# Autodesk Inventor assembly: radio on stand
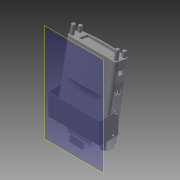
[picture p0: Inventor's stored thumbnail of the model, 180x180]
Saved by Autodesk Inventor 2014 (Build 180170000, 170)
## iProperties
Created: 2014-04-06
Part Number: radio on stand
Document SubType Name: Assembly
Designer: Tyler
Author: Tyler
## Documents named in this file (6)
- C:\Users\Tyler\Documents\ft8900cad\radio on stand.iam
- C:\Users\Tyler\Documents\ft8900cad\radio_base.ipt
- C:\Users\Tyler\Documents\ft8900cad\radio.ipt
- C:\Users\Tyler\Documents\Inventor\Content Center Files\R2014\en-US\GB_T 2671.1-2004\Screw GB_T 2171.1 M4 x 6.ipt
- C:\Users\Tyler\Documents\ft8900cad\controlunit.iam
- C:\Users\Tyler\Documents\ft8900cad\radio_head.ipt
## Components (8 placed, 5 different names)
1. radio_base:1 — Insert:1, Insert:2, Insert:3, Insert:4, Insert:5, Insert:6, Mate:2, Flush:3, Flush:4
2. radio:1 — Insert:1, Insert:2, Mate:1, Flush:1, Flush:2
3. Screw GB/T 2671.1-2004 M4x6 Property Class 4.8:1 — Insert:3
4. Screw GB/T 2671.1-2004 M4x6 Property Class 4.8:2 — Insert:4
5. Screw GB/T 2671.1-2004 M4x6 Property Class 4.8:3 — Insert:5
6. Screw GB/T 2671.1-2004 M4x6 Property Class 4.8:4 — Insert:6
7. controlunit:1 [sub-assembly] — Mate:1, Flush:1, Flush:2, Mate:3, Flush:5, Flush:6
8. radio_head:1 — Mate:3, Flush:5, Flush:6
## Relationships (15: Insert 6, Flush 6, Mate 3)
- Insert:1: radio_base:1 ↔ radio:1
- Insert:2: radio_base:1 ↔ radio:1
- Insert:3: radio_base:1 ↔ Screw GB/T 2671.1-2004 M4x6 Property Class 4.8:1
- Insert:4: radio_base:1 ↔ Screw GB/T 2671.1-2004 M4x6 Property Class 4.8:2
- Insert:5: radio_base:1 ↔ Screw GB/T 2671.1-2004 M4x6 Property Class 4.8:3
- Insert:6: radio_base:1 ↔ Screw GB/T 2671.1-2004 M4x6 Property Class 4.8:4
- Mate:1: radio:1 ↔ controlunit:1
- Flush:1: radio:1 ↔ controlunit:1
- Flush:2: radio:1 ↔ controlunit:1
- Mate:2: radio_base:1
- Flush:3: radio_base:1
- Flush:4: radio_base:1
- Mate:3: controlunit:1 ↔ radio_head:1
- Flush:5: controlunit:1 ↔ radio_head:1
- Flush:6: controlunit:1 ↔ radio_head:1
